# Autodesk Inventor assembly: Ensamblajekight mediom 1.2
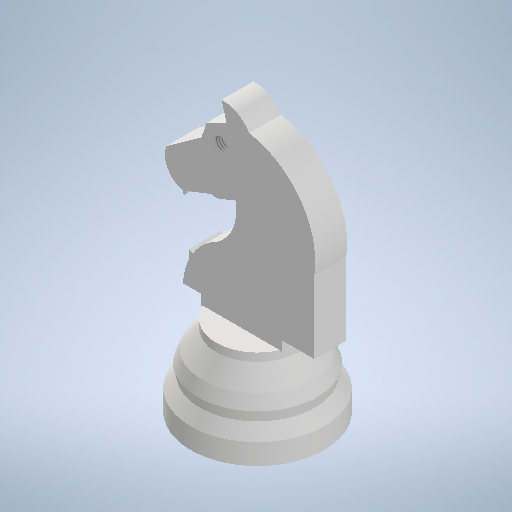
[picture p0: Inventor's stored thumbnail of the model, 512x512]
Saved by Autodesk Inventor 2025.1 (Build 291241000, 241)
## iProperties
Created: 2024-11-01
Part Number: Ensamblajekight mediom 1.2
Document SubType Name: Assembly
Designer: Octavio
Author: Octavio
## Documents named in this file (3)
- C:\Users\Octavio\Documents\Inventor\CABALLO\Ensamblaje knight medium\Ensamblajekight mediom 1.2.iam
- C:\Users\Octavio\Documents\Inventor\CABALLO\Knght 1.0\KIGTH TOP abrebotella medium 1.1.ipt
- C:\Users\Octavio\Documents\Inventor\CABALLO\Knght 1.0\KINGHT BASE  medieum 1.0.ipt
## Components (2 placed, 2 different names)
1. KIGTH TOP abrebotella medium 1.1:1 — Rígido:1
2. KINGHT BASE  medieum 1.0:1 — Rígido:1
## Relationships (1: WeldJoint 1)
- Rígido:1 [WeldJoint] (-0.2 mm): KIGTH TOP abrebotella medium 1.1:1 ↔ KINGHT BASE  medieum 1.0:1
